# Autodesk Inventor assembly: ASM_Micron_with_Inner_Guide
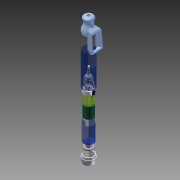
[picture p0: Inventor's stored thumbnail of the model, 180x180]
Saved by Autodesk Inventor 2011 SP2 (Build 150309200, 309)
## iProperties
Created: 2012-01-18
Part Number: ASM_Micron_with_Inner_Guide
Document SubType Name: Assembly
Designer: sungwook
Author: sungwook
## Documents named in this file (17)
- C:\Users\sungwook\Documents\Inventor\Micron20_Base_Tube_Adjst\05222012_Inner_Guide_Tube\ASM_Micron_with_Inner_Guide.iam
- C:\Users\sungwook\Documents\Inventor\Micron20_Base_Tube_Adjst\Parts\Main\Platform_Base_20mm_Rev_old.ipt
- C:\Users\sungwook\Documents\Inventor\Micron20_Base_Tube_Adjst\Parts\Main\Platform_Top_14mm_Rev.ipt
- C:\Users\sungwook\Documents\Inventor\Micron20_Base_Tube_Adjst\Parts\Tool\ASM_Tool_Tip_Rev.iam
- C:\Users\sungwook\Documents\Inventor\Micron20_Base_Tube_Adjst\Assembly\ASM_Motor_Unit_Rev.iam
- C:\Users\sungwook\Documents\Inventor\Micron20_Base_Tube_Adjst\Parts\Main\Eye_Pin_26Ga.ipt
- C:\Users\sungwook\Documents\Inventor\Content Center Files\R2011\en-US\ANSI B18.6.3(12)\ANSI B18.6.3 - 0-80 UNF - 0.1875(15_).ipt
- C:\Users\sungwook\Documents\Inventor\Micron20_Base_Tube_Adjst\Parts\Main\Spring.ipt
- C:\Users\sungwook\Documents\Inventor\Micron20_Base_Tube_Adjst\Parts\ASAP\Handle_ASAP.iam
- C:\Users\sungwook\Documents\Inventor\Micron20_Base_Tube_Adjst\Parts\ASAP\Platform_ASAP.iam
- C:\Users\sungwook\Documents\Inventor\Micron20_Base_Tube_Adjst\Parts\Electronics\PCB_Stack.iam
- C:\Users\sungwook\Documents\Inventor\Micron20_withOldMotor\Parts\Handle\Handle_1_Asm.iam
- C:\Users\sungwook\Documents\Inventor\Micron20_Base_Tube_Adjst\Parts\Handle\Handle_2_Asm.iam
- C:\Users\sungwook\Documents\Inventor\Micron20_Base_Tube_Adjst\Parts\Tool\Tool Mount_Rev.ipt
- C:\Users\sungwook\Documents\Inventor\Micron20_Base_Tube_Adjst\05222012_Inner_Guide_Tube\ss_inner_guide.ipt
- C:\Users\sungwook\Documents\Inventor\Micron20_Base_Tube_Adjst\Parts\Handle\Ver2(Al_RP)\Handle_2_rev2_Asm.iam
- C:\Users\sungwook\Documents\Inventor\Micron20_Base_Tube_Adjst\05222012_Inner_Guide_Tube\inner_guide_asm.iam
## Components (31 placed, 16 different names)
1. Platform_Base_20mm_Rev_old:1 — Mate:4, Mate:6, Mate:8, Angle:1, Mate:29, Mate:30, Mate:31, Mate:32, Flush:23, Mate:33, Mate:35, Mate:38, Mate:39, Mate:40, Mate:41, Mate:44, Flush:24, Flush:25
2. Platform_Top_14mm_Rev:1 — Mate:1, Mate:2, Mate:3, Mate:4, Mate:5, Mate:7, Angle:1, Mate:9, Mate:10, Angle:2, Mate:18, Mate:58, Mate:65
3. ASM_Tool_Tip_Rev:1 [sub-assembly] — Mate:1, Mate:2, Mate:3, Mate:11
4. Handle_ASAP:1 [sub-assembly] — Flush:1, Mate:29, Mate:30, Mate:31, Mate:38
5. Platform_ASAP:1 [sub-assembly] — Mate:16, Mate:17, Mate:18, Mate:57, Mate:59
6. PCB_Stack:1 [sub-assembly] — Mate:39, Mate:40, Mate:41, Mate:47, Mate:72, Mate:73
7. Handle_1_Asm:1 [sub-assembly] — Mate:42, Mate:43, Mate:44
8. Handle_2_Asm:1 [sub-assembly] — Mate:45, Mate:46, Mate:47, Mate:69
9. Tool Mount_Rev:1 — Mate:57, Mate:58, Mate:59, Mate:65
10. Handle_2_Asm:2 [sub-assembly] — Mate:62, Angle:4
11. ss_inner_guide:1 — Mate:68, Mate:69, Mate:70, Flush:24, Flush:25
12. Handle_2_rev2_Asm:1 [sub-assembly] — Mate:70, Mate:71, Mate:72
13. inner_guide_asm:1 [sub-assembly] — Mate:73, Mate:74
14. ASM_Motor_Unit_Rev:1 [sub-assembly] — Mate:5, Mate:6
15. ASM_Motor_Unit_Rev:2 [sub-assembly] — Mate:7, Mate:8
16. ASM_Motor_Unit_Rev:3 [sub-assembly]
17. ASM_Motor_Unit_Rev:4 [sub-assembly]
18. ASM_Motor_Unit_Rev:5 [sub-assembly]
19. ASM_Motor_Unit_Rev:6 [sub-assembly]
20. Cross Recessed Flat Countersunk Head Machine Screw - Type I - Inch 0-80 x 3/16:1 — Mate:11, Mate:16
21. Cross Recessed Flat Countersunk Head Machine Screw - Type I - Inch 0-80 x 3/16:2
22. Cross Recessed Flat Countersunk Head Machine Screw - Type I - Inch 0-80 x 3/16:3 — Mate:17
23. Eye_Pin_26Ga:1 — Mate:9, Mate:10, Angle:2, Mate:34, Mate:36, Mate:37
24. Spring:1 — Mate:33, Mate:34, Mate:35, Mate:36, Mate:37
25. Eye_Pin_26Ga:4 — Mate:32, Flush:23
26. Eye_Pin_26Ga:5
27. Spring:2
28. Eye_Pin_26Ga:6
29. Eye_Pin_26Ga:7
30. Spring:3
31. Eye_Pin_26Ga:8
## Component patterns: (3 elements, first: ASM_Motor_Unit_Rev:1 + ASM_Motor_Unit_Rev:2), Tool Mount Bolts (3 elements), (3 elements, first: Eye_Pin_26Ga:1 + Spring:1 + Eye_Pin_26Ga:4)
## Relationships (52: Mate 45, Flush 4, Angle 3)
- Mate:1: Platform_Top_14mm_Rev:1 ↔ ASM_Tool_Tip_Rev:1
- Mate:2: Platform_Top_14mm_Rev:1 ↔ ASM_Tool_Tip_Rev:1
- Mate:3: Platform_Top_14mm_Rev:1 ↔ ASM_Tool_Tip_Rev:1
- Mate:4: Platform_Base_20mm_Rev_old:1 ↔ Platform_Top_14mm_Rev:1
- Mate:5: Platform_Top_14mm_Rev:1 ↔ ASM_Motor_Unit_Rev:1
- Mate:6: Platform_Base_20mm_Rev_old:1 ↔ ASM_Motor_Unit_Rev:1
- Mate:7: Platform_Top_14mm_Rev:1 ↔ ASM_Motor_Unit_Rev:2
- Mate:8: Platform_Base_20mm_Rev_old:1 ↔ ASM_Motor_Unit_Rev:2
- Angle:1 (180 deg): Platform_Base_20mm_Rev_old:1 ↔ Platform_Top_14mm_Rev:1
- Mate:9: Platform_Top_14mm_Rev:1 ↔ Eye_Pin_26Ga:1
- Mate:10: Platform_Top_14mm_Rev:1 ↔ Eye_Pin_26Ga:1
- Angle:2 (0 deg): Platform_Top_14mm_Rev:1 ↔ Eye_Pin_26Ga:1
- Mate:16: Platform_ASAP:1 ↔ Cross Recessed Flat Countersunk Head Machine Screw - Type I - Inch 0-80 x 3/16:1
- Mate:17: Platform_ASAP:1 ↔ Cross Recessed Flat Countersunk Head Machine Screw - Type I - Inch 0-80 x 3/16:3
- Mate:18: Platform_Top_14mm_Rev:1 ↔ Platform_ASAP:1
- Flush:1: Handle_ASAP:1
- Mate:29 (4.302 mm): Platform_Base_20mm_Rev_old:1 ↔ Handle_ASAP:1
- Mate:30: Platform_Base_20mm_Rev_old:1 ↔ Handle_ASAP:1
- Mate:31: Platform_Base_20mm_Rev_old:1 ↔ Handle_ASAP:1
- Mate:32: Platform_Base_20mm_Rev_old:1 ↔ Eye_Pin_26Ga:4
- Flush:23: Platform_Base_20mm_Rev_old:1 ↔ Eye_Pin_26Ga:4
- Mate:33: Platform_Base_20mm_Rev_old:1 ↔ Spring:1
- Mate:34: Eye_Pin_26Ga:1 ↔ Spring:1
- Mate:35: Platform_Base_20mm_Rev_old:1 ↔ Spring:1
- Mate:36: Eye_Pin_26Ga:1 ↔ Spring:1
- Mate:37: Eye_Pin_26Ga:1 ↔ Spring:1
- Mate:38: Platform_Base_20mm_Rev_old:1 ↔ Handle_ASAP:1
- Mate:39: Platform_Base_20mm_Rev_old:1 ↔ PCB_Stack:1
- Mate:40: Platform_Base_20mm_Rev_old:1 ↔ PCB_Stack:1
- Mate:41: Platform_Base_20mm_Rev_old:1 ↔ PCB_Stack:1
- Mate:42: Handle_1_Asm:1
- Mate:43: Handle_1_Asm:1
- Mate:44: Platform_Base_20mm_Rev_old:1 ↔ Handle_1_Asm:1
- Mate:45: Handle_2_Asm:1
- Mate:46: Handle_2_Asm:1
- Mate:47: PCB_Stack:1 ↔ Handle_2_Asm:1
- Mate:57: Platform_ASAP:1 ↔ Tool Mount_Rev:1
- Mate:58: Platform_Top_14mm_Rev:1 ↔ Tool Mount_Rev:1
- Mate:59: Platform_ASAP:1 ↔ Tool Mount_Rev:1
- Mate:62: Handle_2_Asm:2
- Angle:4 (180 deg): Handle_2_Asm:2
- Mate:65: Platform_Top_14mm_Rev:1 ↔ Tool Mount_Rev:1
- Mate:68: ss_inner_guide:1
- Mate:69: Handle_2_Asm:1 ↔ ss_inner_guide:1
- Mate:70: ss_inner_guide:1 ↔ Handle_2_rev2_Asm:1
- Mate:71: Handle_2_rev2_Asm:1
- Mate:72: PCB_Stack:1 ↔ Handle_2_rev2_Asm:1
- Flush:24: Platform_Base_20mm_Rev_old:1 ↔ ss_inner_guide:1
- Flush:25: Platform_Base_20mm_Rev_old:1 ↔ ss_inner_guide:1
- Mate:73: PCB_Stack:1 ↔ inner_guide_asm:1
- Mate:74: inner_guide_asm:1
- Mate:11: ASM_Tool_Tip_Rev:1 ↔ Cross Recessed Flat Countersunk Head Machine Screw - Type I - Inch 0-80 x 3/16:1
